# Autodesk Inventor assembly: Assembly 2017_08_23
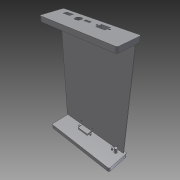
[picture p0: Inventor's stored thumbnail of the model, 180x180]
Saved by Autodesk Inventor 2012 (Build 160160000, 160)
## iProperties
Created: 2017-04-26
Part Number: Assembly 2017_08_23
Document SubType Name: Assembly
Designer: Brandon
Author: Brandon
## Documents named in this file (11)
- C:\Users\Brandon\Dropbox\Admiral Instruments Dropbox\Squidstat Plus 2.0 (single channel, with EIS)\Enclosure\Assembly 2017_08_23.iam
- C:\Users\Brandon\Dropbox\Admiral Instruments Dropbox\Squidstat Plus 2.0 (single channel, with EIS)\Enclosure\PCB.ipt
- C:\Users\Brandon\Dropbox\Admiral Instruments Dropbox\Squidstat Plus 2.0 (single channel, with EIS)\Enclosure\LED on indicator.ipt
- C:\Users\Brandon\Dropbox\Admiral Instruments Dropbox\Squidstat Plus 2.0 (single channel, with EIS)\Enclosure\USB A block.ipt
- C:\Users\Brandon\Dropbox\Admiral Instruments Dropbox\Squidstat Plus 2.0 (single channel, with EIS)\Enclosure\Grounded banana jack.ipt
- C:\Users\Brandon\Dropbox\Admiral Instruments Dropbox\Squidstat Plus 2.0 (single channel, with EIS)\Enclosure\back cover.ipt
- C:\Users\Brandon\Dropbox\Admiral Instruments Dropbox\Squidstat Plus 2.0 (single channel, with EIS)\Enclosure\front cover.ipt
- C:\Users\Brandon\Dropbox\Admiral Instruments Dropbox\Squidstat Plus 2.0 (single channel, with EIS)\Enclosure\On-off pushbutton.ipt
- C:\Users\Brandon\Dropbox\Admiral Instruments Dropbox\Squidstat Plus 2.0 (single channel, with EIS)\Enclosure\DB15 connector 2017_06_14.ipt
- C:\Users\Brandon\Dropbox\Admiral Instruments Dropbox\Squidstat Plus 2.0 (single channel, with EIS)\Enclosure\DB9 connector 2017_06_14.ipt
- C:\Users\Brandon\Dropbox\Admiral Instruments Dropbox\Squidstat Plus 2.0 (single channel, with EIS)\Enclosure\Bigger slide switch 2017_06_14.ipt
## Components (10 placed, 10 different names)
1. PCB:1 — Flush:1, Insert:1, Insert:4, Angle:4, Flush:5, Insert:7, Insert:8, Insert:9, Angle:8, Insert:10, Angle:9, Insert:11, Angle:10
2. LED on indicator:1 — Flush:1, Insert:1, Angle:3
3. Grounded banana jack:1 — Insert:4, Angle:4
4. back cover:1 — Mate:3, Mate:4, Flush:4, Flush:5
5. front cover:1 — Flush:3, Mate:2, Flush:4
6. USB A block:1 — Insert:7, Angle:7
7. On-off pushbutton:1 — Insert:8
8. DB15 connector 2017_06_14:1 — Insert:9, Angle:8
9. DB9 connector 2017_06_14:1 — Insert:10, Angle:9
10. Bigger slide switch 2017_06_14:1 — Insert:11, Angle:10
## Relationships (20: Insert 7, Angle 6, Flush 4, Mate 3)
- Flush:1: PCB:1 ↔ LED on indicator:1
- Insert:1: PCB:1 ↔ LED on indicator:1
- Angle:3 (180 deg): LED on indicator:1
- Insert:4: PCB:1 ↔ Grounded banana jack:1
- Angle:4 (0 deg): PCB:1 ↔ Grounded banana jack:1
- Flush:3 (114.3 mm): front cover:1
- Mate:2: front cover:1
- Mate:3 (114.3 mm): back cover:1
- Mate:4: back cover:1
- Flush:4: back cover:1 ↔ front cover:1
- Flush:5 (7.2898 mm): PCB:1 ↔ back cover:1
- Insert:7: PCB:1 ↔ USB A block:1
- Angle:7 (180 deg): USB A block:1
- Insert:8: PCB:1 ↔ On-off pushbutton:1
- Insert:9: PCB:1 ↔ DB15 connector 2017_06_14:1
- Angle:8 (180 deg): PCB:1 ↔ DB15 connector 2017_06_14:1
- Insert:10: PCB:1 ↔ DB9 connector 2017_06_14:1
- Angle:9 (0 deg): PCB:1 ↔ DB9 connector 2017_06_14:1
- Insert:11: PCB:1 ↔ Bigger slide switch 2017_06_14:1
- Angle:10 (0 deg): PCB:1 ↔ Bigger slide switch 2017_06_14:1
